# Autodesk Inventor assembly: BearingMountSingleSupport
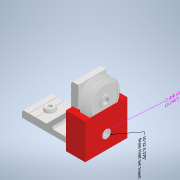
[picture p0: Inventor's stored thumbnail of the model, 180x180]
Saved by Autodesk Inventor 2020.2 (Build 242310000, 310)
## iProperties
Created: 2018-01-10
Part Number: BearingMountSingleSupport
Document SubType Name: Assembly
Designer: robst
Author: robst
Revision Number: ANY
## Documents named in this file (8)
- C:\git\CAD-Development\robSteele\2020LiftMechanism\BearingMountSingleSupport.iam
- C:\git\CAD-Development\robSteele\2020LiftMechanism\REV-21-1203 Preload 2 Screws Assembly.iam
- C:\git\CAD-Development\robSteele\2020LiftMechanism\10-32 Slim Nylock Nut.ipt
- C:\git\CAD-Development\robSteele\2020LiftMechanism\Bearing Delrin Spacer.ipt
- C:\git\CAD-Development\robSteele\2020LiftMechanism\REV-29-1014.ipt
- C:\git\CAD-Development\robSteele\2020LiftMechanism\10-32 1.5 inch Long.ipt
- C:\git\CAD-Development\robSteele\2020LiftMechanism\preventWireJumpingSingleSupport.ipt
- C:\git\CAD-MfgResources\McMaster-Carr\BrassHeatSetInsertForPlastic\10-32 0_375 93365A156_HEAT-SET INSERTS FOR PLASTICS.ipt
## Components (7 placed, 7 different names)
1. REV-21-1203 Preload 2 Screws Assembly_65 [sub-assembly] — Insert:1
2. 10-32 Slim Nylock Nut_66
3. Bearing Delrin Spacer_67
4. REV-29-1014_68
5. 10-32 1.5 inch Long_69
6. preventWireJumpingSingleSupport:1 — Insert:1, Insert:2
7. 10-32 0_375 93365A156_HEAT-SET INSERTS FOR PLASTICS:1 — Insert:2
## Relationships (2: Insert 2)
- Insert:1: REV-21-1203 Preload 2 Screws Assembly_65 ↔ preventWireJumpingSingleSupport:1
- Insert:2: preventWireJumpingSingleSupport:1 ↔ 10-32 0_375 93365A156_HEAT-SET INSERTS FOR PLASTICS:1
